# Autodesk Inventor assembly: 739282
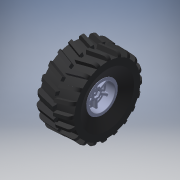
[picture p0: Inventor's stored thumbnail of the model, 180x180]
Saved by Autodesk Inventor 2019 (Build 230136000, 136)
## iProperties
Category: Add-on Components
Company: Autodesk Inc.
Created: 2014-11-26
Part Number: 739282
Document SubType Name: Assembly
Designer: Tetrix
Catalog Web Link: http://www.tetrixrobotics.com/Wheels/TETRIX_All-Terrain_Tire
Vendor: Tetrix
Author: Autodesk Inc.
## Documents named in this file (3)
- C:\Users\tbloo\Documents\Inventor\FTC Tetrix KOP\Miscellaneous\Tetrix_39282.iam
- C:\Users\tbloo\Downloads\FTC Tetrix KOP\Miscellaneous\Tetrix_39282_Hub.ipt
- C:\Users\tbloo\Downloads\FTC Tetrix KOP\Miscellaneous\Tetrix_39282_Tire.ipt
## Components (2 placed, 2 different names)
1. Tetrix_39282_Hub:1 — Insert:1
2. Tetrix_39282_Tire:1 — Insert:1
## Relationships (1: Insert 1)
- Insert:1: Tetrix_39282_Hub:1 ↔ Tetrix_39282_Tire:1
